# Autodesk Inventor assembly: MBRDAC23-2-8
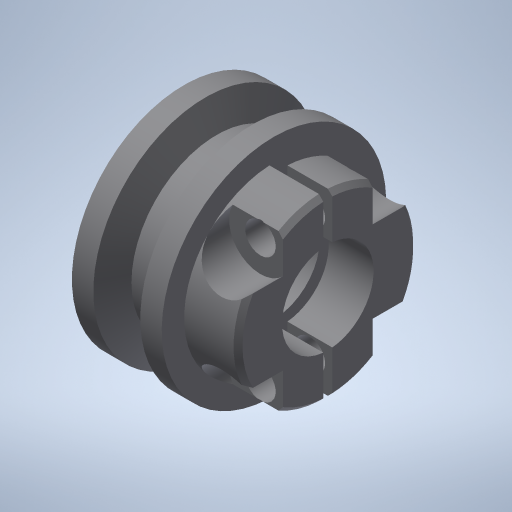
[picture p0: Inventor's stored thumbnail of the model, 512x512]
Saved by Autodesk Inventor 2024 (Build 280153000, 153)
## iProperties
Created: 2024-03-05
Part Number: MBRDAC23-2-8
Catalog Web Link: www.cadenas.de
Description: MBRDC, MBRDAC-Pulleys for Round Belts - Clamping Type - Trapezoid Groove
Vendor: MISUMI
Document SubType Name: Assembly
Designer: psAdmin
Manufacturer: MISUMI
Mass: 4.87159 g
Surface Area: 34.0443 cm^2
Volume: 4.87159 cm^3
Density: 1 g/cm^3
Category: PARTsolutions
Company: MISUMI
PSOL_IDENT_0: {$CADENAS_DATA/23d-libs/misumi/metric/52_belts_pulleys/mbrdc_asmtab.prj},201 {VTYP=3D},{STYP=ASSTAB}
PSOL_IDENT_1: ,{NB=MBRDAC23-2-8},{LINA=MBRDAC23-2-8},{NN=MBRDC, MBRDAC},{DATE=06.06.2021 23:11:25},{GEOMDATE=16.06
PSOL_IDENT_2: .2016 00:32:00},{VERSION=},{LINEID=30},{WBVAR=MAT,PD,DDS},{WBNUMERIC=PD,DDS}  {NB=MBRDAC23-2-8},{LIN
PSOL_IDENT_3: A=MBRDAC23-2-8},{KT=DUMMY},{PN=MBRDAC23-2-8},{TYPE=MBRDAC},{MAT=2},{ST=Clear Anodizing},{AC=Hexagon
PSOL_IDENT_4: Socket Head Cap Screw (x2) Stainless Steel},{PD=23},{PD0=23,28,30,40,45,48,60,80},{U=2.0},{DDS=8.00}
PSOL_IDENT_5: ,{DS0=5,6,6.35,8},{D=20},{D1=25},{D2=19},{HH=2.0},{W=4.4},{L=16},{T=10},{LL=2.5},{X=7.0},{Y=3.5},{M=
PSOL_IDENT_6: M3},{CBD=4},{MM=3.000},{MMMIN=2.459},{DD1=6.5},{DD2=3.5},{PPATH=mbrdc/mbrdc_asmtpl.prj}
NB: MBRDAC23-2-8
NN: MBRDC, MBRDAC
NT: Pulleys for Round Belts - Clamping Type - Trapezoid Groove
NBSYN: $PN.
LINA: MBRDAC23-2-8
CATALOG: Misumi
PN: MBRDAC23-2-8
MAT: A5052
ST: Clear Anodizing
AC: Hexagon Socket Head Cap Screw (x2) Stainless Steel
PD: 23
U: 2
DDS: 8
D: 20
D1: 25
D2: 19
HH: 2
W: 4.4
L: 16
T: 10
LL: 2.5
X: 7
Y: 3.5
M: M3
CBD: 4
SUPPLIER: MISUMI
ARTICLENO: MBRDAC23-2-8
BOMINFO: MBRDAC23-2-8
CREATOR: CADENAS GmbH
Title: MBRDAC23-2-8
Author: Cadenas PARTsolutions
Comments: Pulleys for Round Belts - Clamping Type - Trapezoid Groove
## Documents named in this file (4)
- C:\Users\haruy\OneDrive - Kyushu University\KURT_工房共有\2023~2024\ハード\CAD\2024NHK\000_parts\タイミングベルト\circileberut\AIS2024\MBRDAC23-2-8.iam
- C:\Users\haruy\OneDrive - Kyushu University\KURT_工房共有\2023~2024\ハード\CAD\2024NHK\000_parts\タイミングベルト\circileberut\AIS2024\MBRDAC23-2-8_p1.ipt
- C:\Users\haruy\OneDrive - Kyushu University\KURT_工房共有\2023~2024\ハード\CAD\2024NHK\000_parts\タイミングベルト\circileberut\AIS2024\MBRDAC23-2-8_p2.ipt
- C:\Users\haruy\OneDrive - Kyushu University\KURT_工房共有\2023~2024\ハード\CAD\2024NHK\000_parts\タイミングベルト\circileberut\AIS2024\M3x8_p3.ipt
## Components (4 placed, 3 different names)
1. MBRDAC23-2-8_p1:1 — part1_to_part2_Z@1 <-> part2_to_part1_Z@2
2. MBRDAC23-2-8_p2:1 — part1_to_part2_Z@1 <-> part2_to_part1_Z@2, part2_to_screw1_Z@2 <-> IP1_Z@3, part2_to_screw2_Z@2 <-> IP1_Z@4
3. M3x8_p3:1 — part2_to_screw1_Z@2 <-> IP1_Z@3
4. M3x8_p3:2 — part2_to_screw2_Z@2 <-> IP1_Z@4
## Relationships (3: Mate 3)
- part1_to_part2_Z@1 <-> part2_to_part1_Z@2 [Mate]: MBRDAC23-2-8_p1:1 ↔ MBRDAC23-2-8_p2:1
- part2_to_screw1_Z@2 <-> IP1_Z@3 [Mate]: MBRDAC23-2-8_p2:1 ↔ M3x8_p3:1
- part2_to_screw2_Z@2 <-> IP1_Z@4 [Mate]: MBRDAC23-2-8_p2:1 ↔ M3x8_p3:2
